# Autodesk Inventor assembly: 240614_체인
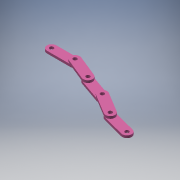
[picture p0: Inventor's stored thumbnail of the model, 180x180]
Saved by Autodesk Inventor 2016 (Build 200138000, 138)
## iProperties
Created: 2024-06-14
Part Number: 240614_체인
Material: 일반
Document SubType Name: Assembly
Designer: pc
Author: pc
## Documents named in this file (2)
- D:\CAD_HCH\240614\240614_체인.iam
- D:\CAD_HCH\240614\240614_체인1.ipt
## Components (5 placed, 1 different names)
1. 240614_체인1:1 — 메이트:1, 메이트:2
2. 240614_체인1:2 — 메이트:1, 메이트:2, 메이트:3, 메이트:4
3. 240614_체인1:3 — 메이트:3, 메이트:4, 메이트:5, 메이트:6
4. 240614_체인1:4 — 메이트:5, 메이트:6, 메이트:7, 메이트:8
5. 240614_체인1:5 — 메이트:7, 메이트:8
## Relationships (8: Mate 8)
- 메이트:1 [Mate]: 240614_체인1:1 ↔ 240614_체인1:2
- 메이트:2 [Mate]: 240614_체인1:1 ↔ 240614_체인1:2
- 메이트:3 [Mate]: 240614_체인1:2 ↔ 240614_체인1:3
- 메이트:4 [Mate]: 240614_체인1:2 ↔ 240614_체인1:3
- 메이트:5 [Mate]: 240614_체인1:3 ↔ 240614_체인1:4
- 메이트:6 [Mate]: 240614_체인1:3 ↔ 240614_체인1:4
- 메이트:7 [Mate]: 240614_체인1:4 ↔ 240614_체인1:5
- 메이트:8 [Mate]: 240614_체인1:4 ↔ 240614_체인1:5
